# Autodesk Inventor assembly: Link3
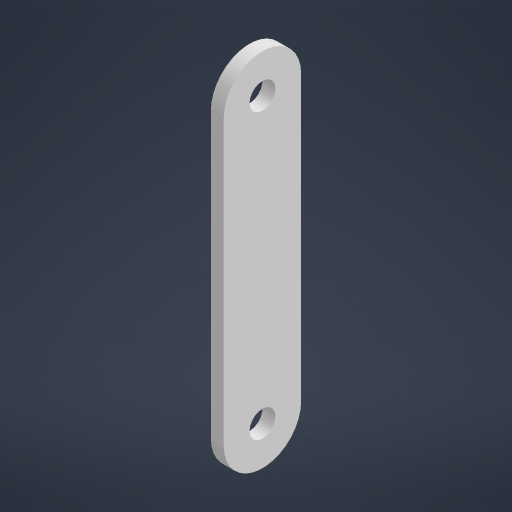
[picture p0: Inventor's stored thumbnail of the model, 512x512]
Saved by Autodesk Inventor 2023 (Build 270158000, 158)
## iProperties
Created: 2023-09-10
Part Number: Link3
Document SubType Name: Assembly
Designer: philo
Author: philo
## Documents named in this file (2)
- C:\Users\philo\OneDrive\Desktop\HK1-2024\TT ROBOT\02_3D_design_new\Link3.iam
- C:\Users\philo\OneDrive\Desktop\HK1-2024\TT ROBOT\02_3D_design_new\Link3Do.ipt
## Components (1 placed, 1 different names)
1. Link3Do:1 — Angle:1
## Relationships (1: Angle 1)
- Angle:1 (0 deg): Link3Do:1
